# Autodesk Inventor assembly: predator mini cam standoff mount
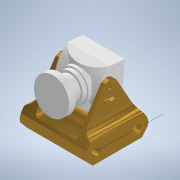
[picture p0: Inventor's stored thumbnail of the model, 180x180]
Saved by Autodesk Inventor 2020 (Build 240168000, 168)
## iProperties
Created: 2022-05-05
Part Number: predator mini cam standoff mount
Document SubType Name: Assembly
Designer: Steven
Author: Steven
## Documents named in this file (3)
- Y:\FPV drone stuff\0 Street League\Frames\PB-Kauri-X\3D prints\35 mm canopy\predator mini cam standoff mount.iam
- Y:\FPV drone stuff\0 Street League\Frames\PB-Kauri-X\3D prints\35 mm canopy\mini predator dummy camera.ipt
- Y:\FPV drone stuff\0 Street League\Frames\PB-Kauri-X\3D prints\35 mm canopy\Kauri camera predator mini standoff mount.ipt
## Components (2 placed, 2 different names)
1. mini predator dummy camera:1 — Insert:1
2. Kauri camera predator mini standoff mount:1 — Insert:1, Mate:1
## Relationships (2: Insert 1, Mate 1)
- Insert:1: mini predator dummy camera:1 ↔ Kauri camera predator mini standoff mount:1
- Mate:1: Kauri camera predator mini standoff mount:1
